# Autodesk Inventor assembly: WheelAssembly_v8
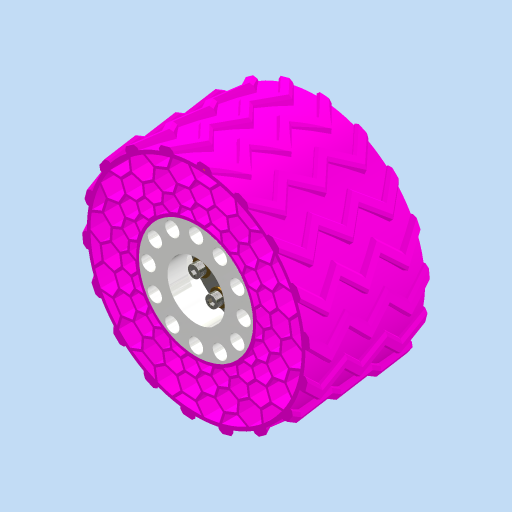
[picture p0: Inventor's stored thumbnail of the model, 512x512]
Saved by Autodesk Inventor 2023 (Build 270158000, 158)
## iProperties
Created: 2023-04-06
Part Number: WheelAssembly_v8
Document SubType Name: Assembly
Designer: asach
Mass: 719.998 g
Surface Area: 4242.43 cm^2
Volume: 481.212 cm^3
Density: 1.49622 g/cm^3
Author: asach
## Documents named in this file (7)
- C:\Github\BehrendURC\CAD\Chassis V3\Wheel\WheelAssembly_v8.iam
- C:\Github\BehrendURC\CAD\Chassis V3\Wheel\Tire_v8.ipt
- C:\Github\BehrendURC\CAD\Chassis V3\Wheel\ThickWheelPlate_v8.ipt
- C:\Github\BehrendURC\CAD\Chassis V3\Wheel\WheelPlateBolt_1inch.ipt
- C:\Github\BehrendURC\CAD\Chassis V3\Wheel\Washer.ipt
- C:\Github\BehrendURC\CAD\Chassis V3\Wheel\WheelPlateNut.ipt
- C:\Projects\FlexibleWheel\HubCap_v7.ipt
## Components (53 placed, 6 different names)
1. Tire_v8:1 — Mate:1, Mate:2, Mate:3, Mate:4, Mate:5, Mate:6, Mate:7, Mate:16, Mate:19
2. ThickWheelPlate_v8:1 — Mate:1, Mate:2, Mate:3, Mate:10, Mate:15
3. ThickWheelPlate_v8:2 — Mate:4, Mate:5, Mate:6, Mate:12, Mate:14, Mate:18
4. HubCap_v7:1 — Mate:15, Mate:16, Mate:17
5. HubCap_v7:2 — Mate:18, Mate:19, Mate:20
6. Washer:2 — Mate:11, Mate:12, Mate:20
7. Washer:1 — Mate:8, Mate:9, Mate:10
8. WheelPlateBolt_1inch:1 — Mate:7, Mate:8, Mate:9, Mate:11, Mate:13
9. WheelPlateNut:1 — Mate:13, Mate:14
10. Washer:3
11. Washer:4
12. WheelPlateBolt_1inch:2
13. WheelPlateNut:2
14. Washer:5
15. Washer:6
16. WheelPlateBolt_1inch:3 — Mate:17
17. WheelPlateNut:3
18. Washer:7
19. Washer:8
20. WheelPlateBolt_1inch:4
21. WheelPlateNut:4
22. Washer:9
23. Washer:10
24. WheelPlateBolt_1inch:5
25. WheelPlateNut:5
26. Washer:11
27. Washer:12
28. WheelPlateBolt_1inch:6
29. WheelPlateNut:6
30. Washer:13
31. Washer:14
32. WheelPlateBolt_1inch:7
33. WheelPlateNut:7
34. Washer:15
35. Washer:16
36. WheelPlateBolt_1inch:8
37. WheelPlateNut:8
38. Washer:17
39. Washer:18
40. WheelPlateBolt_1inch:9
41. WheelPlateNut:9
42. Washer:19
43. Washer:20
44. WheelPlateBolt_1inch:10
45. WheelPlateNut:10
46. Washer:21
47. Washer:22
48. WheelPlateBolt_1inch:11
49. WheelPlateNut:11
50. Washer:23
51. Washer:24
52. WheelPlateBolt_1inch:12
53. WheelPlateNut:12
## Component patterns: (12 elements, first: Washer:2 + Washer:1 + WheelPlateBolt_1inch:1 + WheelPlateNut:1)
## Relationships (20: Mate 20)
- Mate:1: Tire_v8:1 ↔ ThickWheelPlate_v8:1
- Mate:2: Tire_v8:1 ↔ ThickWheelPlate_v8:1
- Mate:3: Tire_v8:1 ↔ ThickWheelPlate_v8:1
- Mate:4: Tire_v8:1 ↔ ThickWheelPlate_v8:2
- Mate:5: Tire_v8:1 ↔ ThickWheelPlate_v8:2
- Mate:6: Tire_v8:1 ↔ ThickWheelPlate_v8:2
- Mate:7: Tire_v8:1 ↔ WheelPlateBolt_1inch:1
- Mate:8: Washer:1 ↔ WheelPlateBolt_1inch:1
- Mate:9: Washer:1 ↔ WheelPlateBolt_1inch:1
- Mate:10: ThickWheelPlate_v8:1 ↔ Washer:1
- Mate:11: Washer:2 ↔ WheelPlateBolt_1inch:1
- Mate:12: ThickWheelPlate_v8:2 ↔ Washer:2
- Mate:13: WheelPlateBolt_1inch:1 ↔ WheelPlateNut:1
- Mate:14: ThickWheelPlate_v8:2 ↔ WheelPlateNut:1
- Mate:15: ThickWheelPlate_v8:1 ↔ HubCap_v7:1
- Mate:16: Tire_v8:1 ↔ HubCap_v7:1
- Mate:17: HubCap_v7:1 ↔ WheelPlateBolt_1inch:3
- Mate:18: ThickWheelPlate_v8:2 ↔ HubCap_v7:2
- Mate:19: Tire_v8:1 ↔ HubCap_v7:2
- Mate:20: HubCap_v7:2 ↔ Washer:2
